# Autodesk Inventor assembly: Assembly
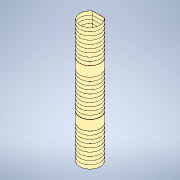
[picture p0: Inventor's stored thumbnail of the model, 180x180]
Saved by Autodesk Inventor 2021 (Build 250183000, 183)
## iProperties
Created: 2020-05-28
Part Number: Assembly
Document SubType Name: Assembly
Designer: aydan
Author: aydan
## Documents named in this file (3)
- C:\Users\aydan\OneDrive\Documents\Inventor\Garcia_Lab\Altuntas_Engine\Assembly.iam
- C:\Users\aydan\OneDrive\Documents\Inventor\Garcia_Lab\Altuntas_Engine\Small_Ring.ipt
- C:\Users\aydan\OneDrive\Documents\Inventor\Garcia_Lab\Altuntas_Engine\Large_Ring.ipt
## Components (30 placed, 2 different names)
1. Small_Ring:1 — Mate:1
2. Small_Ring:2 — Mate:1, Mate:2
3. Small_Ring:3 — Mate:2, Mate:3
4. Small_Ring:4 — Mate:3, Mate:4
5. Small_Ring:5 — Mate:4, Mate:5
6. Small_Ring:6 — Mate:8, Mate:9
7. Small_Ring:7 — Mate:5, Mate:6
8. Small_Ring:8 — Mate:7, Mate:8
9. Small_Ring:9 — Mate:6, Mate:7
10. Large_Ring:1 — Mate:9, Mate:19
11. Small_Ring:10 — Mate:20
12. Small_Ring:11
13. Small_Ring:12
14. Small_Ring:13
15. Small_Ring:14
16. Small_Ring:15 — Mate:29
17. Small_Ring:16
18. Small_Ring:17
19. Small_Ring:18
20. Small_Ring:19 — Mate:19, Mate:20
21. Small_Ring:20 — Mate:30
22. Small_Ring:21
23. Small_Ring:22
24. Small_Ring:23
25. Small_Ring:24
26. Small_Ring:25
27. Small_Ring:26
28. Small_Ring:27
29. Small_Ring:28
30. Large_Ring:3 — Mate:29, Mate:30
## Relationships (29: Mate 29)
- Mate:1: Small_Ring:1 ↔ Small_Ring:2
- Mate:2: Small_Ring:2 ↔ Small_Ring:3
- Mate:3: Small_Ring:3 ↔ Small_Ring:4
- Mate:4: Small_Ring:4 ↔ Small_Ring:5
- Mate:5: Small_Ring:5 ↔ Small_Ring:7
- Mate:6: Small_Ring:7 ↔ Small_Ring:9
- Mate:7: Small_Ring:8 ↔ Small_Ring:9
- Mate:8: Small_Ring:6 ↔ Small_Ring:8
- Mate:9: Small_Ring:6 ↔ Large_Ring:1
- [Mate]: Small_Ring:10 ↔ Small_Ring:11
- [Mate]: Small_Ring:11 ↔ Small_Ring:12
- [Mate]: Small_Ring:12 ↔ Small_Ring:13
- [Mate]: Small_Ring:13 ↔ Small_Ring:14
- [Mate]: Small_Ring:14 ↔ Small_Ring:16
- [Mate]: Small_Ring:16 ↔ Small_Ring:18
- [Mate]: Small_Ring:17 ↔ Small_Ring:18
- [Mate]: Small_Ring:15 ↔ Small_Ring:17
- Mate:19: Large_Ring:1 ↔ Small_Ring:19
- Mate:20: Small_Ring:10 ↔ Small_Ring:19
- [Mate]: Small_Ring:20 ↔ Small_Ring:21
- [Mate]: Small_Ring:21 ↔ Small_Ring:22
- [Mate]: Small_Ring:22 ↔ Small_Ring:23
- [Mate]: Small_Ring:23 ↔ Small_Ring:24
- [Mate]: Small_Ring:24 ↔ Small_Ring:26
- [Mate]: Small_Ring:26 ↔ Small_Ring:28
- [Mate]: Small_Ring:27 ↔ Small_Ring:28
- [Mate]: Small_Ring:25 ↔ Small_Ring:27
- Mate:29: Small_Ring:15 ↔ Large_Ring:3
- Mate:30: Small_Ring:20 ↔ Large_Ring:3
## Named parameters: d9_d0 = 0 mm, d11_d1 = 0 mm, d12_d2 = 0 mm, d13_d3 = 0 mm, d14_d4 = 0 mm, d15_d5 = 0 mm, d16_d6 = 0 mm, d17_d7 = 0 mm, d20_d0 = 0 mm, d22_d1 = 0 mm, d23_d2 = 0 mm, d24_d3 = 0 mm, d25_d4 = 0 mm, d26_d5 = 0 mm, d27_d6 = 0 mm, d28_d7 = 0 mm
